# Autodesk Inventor assembly: .
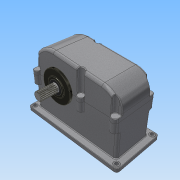
[picture p0: Inventor's stored thumbnail of the model, 180x180]
Saved by Autodesk Inventor 2020.1 (Build 241239000, 239)
## iProperties
Shininess: 64.0
Length Units: 11269
Angle Units: 11279
Time Units: 11290
Mass Units: 11283
Length Display Precision: 3
Angle Display Precision: 2
Compacted: True
+MSCProtocol1+ProtocolID: P00031106203922045
+MSCProtocol2+Protocol: P00031106203922045<@PID>[Version]<@EL>Version=2.2<@EL>[BaseView]<@EL>UpdateAll=0<@EL>[Main]<@EL>DataFile=SpiData|asmpart<@EL>View=MODEL<@EL>[View]<@EL>Data=(setq _data (list "0"))<@EL>Driver=C:/PROGRAM FILES/MECHSOFT/MSINVENTOR7/DATA/DRV/USERPART.LSP<@EL>View=MODEL<@EL>[Object]<@EL>Description=Assembly protocol<@EL>CADDescription=GearBox.iam<@EL>ProtID=P00031106203922045<@EL>[Files]<@EL>Output=C:\DOCUME~1\ales\LOCALS~1\Temp\P00031106203922045.bmp<@EL>[Globals]<@EL>Path=C:\PROGRAM FILES\MECHSOFT\MSINVENTOR7\DATA\<@EL>Caption=Assembly protocol<@EL>NormName=Assembly protocol<@EL>DataChanged=1<@EL>TypeOfPart=10<@EL>Model=Asmpart<@EL>Language=NO<@EL>PrfStd=ISO<@EL>Standard=ISO<@EL>Changed=0<@EL>OldModelId=Asmpart<@EL>Bom7=1<@EL>OwnerHWND=9242094<@EL>BOM5=<@EL>BOM6=<@EL>[Acad]<@EL>modelfilename=C:\#demo\MechSoft\Inventor\PowerTrain\GearBox.iam<@EL>SmartPart=1<@EL>ReallySmartPart=1<@EL>FromCad=1<@EL>Drawn=1<@EL>CADVars=<@EL>Loop=0<@EL>Optim=0<@EL>[Data]<@EL>MSP_PP_MomXX=23.960797{ND<@EL>MSP_PP_Area=613697.07{ND<@EL>MSP_PP_CenterOfMassX=218.76994{ND<@EL>MSP_PP_CenterOfMassY=-46.187597{ND<@EL>MSP_PP_CenterOfMassZ=144.44439{ND<@EL>MSP_PP_Volume=2911533.2{ND<@EL>MSP_PP_Mass=0.0059564747{ND<@EL>MSP_PP_MomYY=38.765179{ND<@EL>MSP_PP_MomZZ=34.054661{ND<@EL>MSP_PP_MomXY=-1.254635{ND<@EL>MSP_PP_MomXZ=-0.57252022{ND<@EL>MSP_PP_MomYZ=-3.1804086{ND<@EL>MSP_PP_PrincMomL1=23.782416{ND<@EL>MSP_PP_PrincMomL2=40.413135{ND<@EL>MSP_PP_PrincMomL3=32.585087{ND<@EL>[GroupMan]<@EL>PosX=58<@EL>PosY=12<@EL>
Created: 2003-11-06
Part Number: .
Document SubType Name: Assembly
Manufacturer: Standard
Standards Organization: Custom
Description: GearBox.iam.
Density: 0.0
Volumn: 0.0
Area: 0.0
PropertySet Name: Model Information
Control State: 0
Master: False
Checked Out: False
## Documents named in this file (17)
- C:\Users\thom_tremblay\Desktop\Inventor ACP Data\Gear Box.iam
- C:\Users\thom_tremblay\Desktop\Inventor ACP Data\Parts\CoverInput.ipt
- C:\Users\thom_tremblay\Desktop\Inventor ACP Data\Parts\CoverOutput.ipt
- C:\Users\thom_tremblay\Desktop\Inventor ACP Data\Parts\GearBoxBottom.ipt
- C:\Users\thom_tremblay\Desktop\Inventor ACP Data\Parts\GearBoxTop.ipt
- C:\Users\thom_tremblay\Desktop\Inventor ACP Data\Parts\BaldorMotorLean.ipt
- C:\Users\thom_tremblay\Desktop\Inventor ACP Data\Parts\Design Accelerator\Shaft1.iam
- C:\Users\thom_tremblay\Desktop\Inventor ACP Data\Parts\Design Accelerator\Shaft2.iam
- C:\Users\thom_tremblay\Desktop\Inventor ACP Data\Gear Box\Design Accelerator\Bearing1.iam
- C:\Users\thom_tremblay\Desktop\Inventor ACP Data\Gear Box\Design Accelerator\Bearing2.iam
- C:\Users\thom_tremblay\Desktop\Inventor ACP Data\Content Center\en-US\BS 1399(1)\BS 1399_ Part 1 - 22359(1).ipt
- C:\Users\thom_tremblay\Desktop\Inventor ACP Data\Gear Box\Design Accelerator\Involute Spline Connection1.iam
- C:\Users\thom_tremblay\Desktop\Inventor ACP Data\Content Center\en-US\BS 1399(1)\BS 1399_ Part 1 - 22329(1).ipt
- C:\Users\thom_tremblay\Desktop\Inventor ACP Data\Gear Box\Design Accelerator\Bearing3.iam
- C:\Users\thom_tremblay\Desktop\Inventor ACP Data\Gear Box\Design Accelerator\Bearing4.iam
- C:\Users\thom_tremblay\Desktop\Inventor ACP Data\Gear Box\Design Accelerator\Involute Spline Connection2.iam
- C:\Users\thom_tremblay\Desktop\Inventor ACP Data\Gear Box\Design Accelerator\Spur Gears1.iam
## Components (15 placed, 10 different names)
1. GearBoxBottom:1 — Flush:1, Flush:2, Mate:1, Flush:3, Flush:4, Mate:2, Mate:3, Mate:4, Mate:5, Mate:6, Mate:7, Insert:1, Insert:2, Flush:6
2. GearBoxTop:1 — Flush:1, Flush:2, Mate:1, Flush:3, Flush:4, Mate:2, Mate:3
3. CoverInput:1 — Mate:4, Mate:5, Rotational:3, Mate:11
4. CoverOutput:1 — Mate:6, Mate:7, Rotational:2, Rigid:1
5. Shaft:2 [sub-assembly] — Insert:1, Mate:8, Flush:5, Mate:14
6. Shaft:3 [sub-assembly] — Insert:2, Mate:9, Mate:10, Mate:12, Mate:13
7. Bearing:1 [sub-assembly] — Mate:8, Flush:5
8. Bearing:3 [sub-assembly] — Rotational:2
9. Involute Spline Connection:1 [sub-assembly]
10. Bearing:4 [sub-assembly] — Mate:9, Flush:6
11. Bearing:5 [sub-assembly] — Mate:10, Mate:11
12. BS 1399 : Part 1 Semi-Dual 22329:1 — Rotational:3
13. BS 1399 : Part 1 Semi-Dual 22359:1 — Rigid:1
14. Involute Spline Connection:2 [sub-assembly]
15. Spur Gears:1 [sub-assembly] — Mate:12, Mate:13, Mate:14
## Relationships (25: Mate 14, Flush 6, Insert 2, RevoluteJoint 2, WeldJoint 1)
- Flush:1: GearBoxBottom:1 ↔ GearBoxTop:1
- Flush:2: GearBoxBottom:1 ↔ GearBoxTop:1
- Mate:1: GearBoxBottom:1 ↔ GearBoxTop:1
- Flush:3: GearBoxBottom:1 ↔ GearBoxTop:1
- Flush:4: GearBoxBottom:1 ↔ GearBoxTop:1
- Mate:2: GearBoxBottom:1 ↔ GearBoxTop:1
- Mate:3: GearBoxBottom:1 ↔ GearBoxTop:1
- Mate:4: GearBoxBottom:1 ↔ CoverInput:1
- Mate:5: GearBoxBottom:1 ↔ CoverInput:1
- Mate:6: GearBoxBottom:1 ↔ CoverOutput:1
- Mate:7: GearBoxBottom:1 ↔ CoverOutput:1
- Insert:1: GearBoxBottom:1 ↔ Shaft:2
- Insert:2: GearBoxBottom:1 ↔ Shaft:3
- Mate:8: Shaft:2 ↔ Bearing:1
- Flush:5: Shaft:2 ↔ Bearing:1
- Rotational:2 [RevoluteJoint]: CoverOutput:1 ↔ Bearing:3
- Rigid:1 [WeldJoint]: CoverOutput:1 ↔ BS 1399 : Part 1 Semi-Dual 22359:1
- Rotational:3 [RevoluteJoint]: CoverInput:1 ↔ BS 1399 : Part 1 Semi-Dual 22329:1
- Mate:9: Shaft:3 ↔ Bearing:4
- Flush:6: GearBoxBottom:1 ↔ Bearing:4
- Mate:10: Shaft:3 ↔ Bearing:5
- Mate:11: CoverInput:1 ↔ Bearing:5
- Mate:12: Shaft:3 ↔ Spur Gears:1
- Mate:13: Shaft:3 ↔ Spur Gears:1
- Mate:14: Shaft:2 ↔ Spur Gears:1
